# Autodesk Inventor assembly: Opaque Base Light Pipe
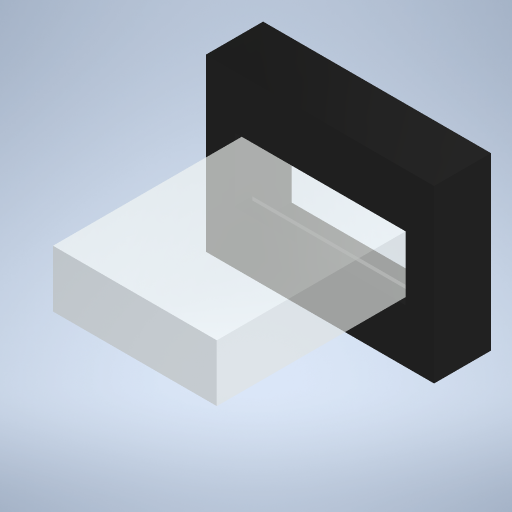
[picture p0: Inventor's stored thumbnail of the model, 512x512]
Saved by Autodesk Inventor 2024 (Build 280153000, 153)
## iProperties
Created: 2024-06-30
Part Number: Opaque Base Light Pipe
Document SubType Name: Assembly
Designer: adam
Author: adam
## Documents named in this file (3)
- C:\Users\adam\Projects\A600KBv2\3dprint\Opaque Base Light Pipe.iam
- C:\Users\adam\Projects\A600KBv2\3dprint\Opaque Rectangular Base.ipt
- C:\Users\adam\Projects\A600KBv2\3dprint\Light Pipe Translucent.ipt
## Components (2 placed, 2 different names)
1. Opaque Rectangular Base:1 — Flush:1
2. Light Pipe Translucent:1 — Flush:1
## Relationships (1: Flush 1)
- Flush:1: Opaque Rectangular Base:1 ↔ Light Pipe Translucent:1
